# Autodesk Inventor assembly: Assembly1
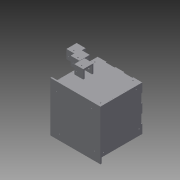
[picture p0: Inventor's stored thumbnail of the model, 180x180]
Saved by Autodesk Inventor 2015 SP1 (Build 190203100, 203)
## iProperties
Created: 2015-08-25
Part Number: Assembly1
Document SubType Name: Assembly
Designer: Kartikye
Author: Kartikye
## Documents named in this file (4)
- C:\Users\Kartikye\Documents\GitHub\SASSat\Structure\V5\Assembly1.iam
- C:\Users\Kartikye\Documents\GitHub\SASSat\Structure\V5\Bottom Panel.ipt
- C:\Users\Kartikye\Documents\GitHub\SASSat\Structure\V5\Side Panel.ipt
- C:\Users\Kartikye\Documents\GitHub\SASSat\Structure\V5\Corner.ipt
## Components (9 placed, 3 different names)
1. Bottom Panel:1 — Flush:8, Mate:3, Mate:4, Mate:5
2. Side Panel:1 — Flush:1, Flush:2, Flush:3, Mate:2
3. Side Panel:2 — Flush:6, Mate:2, Flush:7, Flush:8, Mate:4
4. Side Panel:3 — Mate:1, Flush:4, Flush:5, Flush:6, Flush:7, Mate:3, Mate:6
5. Side Panel:4 — Flush:1, Flush:2, Flush:3, Mate:1, Flush:4, Flush:5, Mate:7
6. Corner:1 — Mate:5, Mate:6, Mate:7
7. Corner:2
8. Corner:3
9. Corner:4
## Relationships (15: Flush 8, Mate 7)
- Flush:1: Side Panel:1 ↔ Side Panel:4
- Flush:2: Side Panel:1 ↔ Side Panel:4
- Flush:3: Side Panel:1 ↔ Side Panel:4
- Mate:1: Side Panel:3 ↔ Side Panel:4
- Flush:4: Side Panel:3 ↔ Side Panel:4
- Flush:5: Side Panel:3 ↔ Side Panel:4
- Flush:6: Side Panel:2 ↔ Side Panel:3
- Mate:2: Side Panel:1 ↔ Side Panel:2
- Flush:7: Side Panel:2 ↔ Side Panel:3
- Flush:8: Bottom Panel:1 ↔ Side Panel:2
- Mate:3: Bottom Panel:1 ↔ Side Panel:3
- Mate:4: Bottom Panel:1 ↔ Side Panel:2
- Mate:5: Bottom Panel:1 ↔ Corner:1
- Mate:6: Side Panel:3 ↔ Corner:1
- Mate:7: Side Panel:4 ↔ Corner:1
